# Autodesk Inventor assembly: spurgearTest
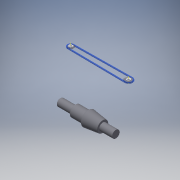
[picture p0: Inventor's stored thumbnail of the model, 180x180]
Saved by Autodesk Inventor 2016 (Build 200138000, 138)
## iProperties
Created: 2016-04-25
Part Number: spurgearTest
Document SubType Name: Assembly
Designer: Henrik Samuelsson
Author: Henrik Samuelsson
## Documents named in this file (4)
- C:\Users\Henrik Samuelsson\Documents\Killer-Bot-2016\AutodeskWorkspace\spurgearTest.iam
- C:\Users\Henrik Samuelsson\Documents\Killer-Bot-2016\AutodeskWorkspace\mountingHub6mm.ipt
- C:\Users\Henrik Samuelsson\Documents\Killer-Bot-2016\AutodeskWorkspace\spurgearTest\Design Accelerator\Shaft1.iam
- C:\Users\Henrik Samuelsson\Documents\Killer-Bot-2016\AutodeskWorkspace\spurgearTest\Design Accelerator\Chain Drive2.iam
## Components (4 placed, 3 different names)
1. mountingHub6mm:1 — Flush:1, Mate:2
2. mountingHub6mm:2 — Flush:1, Mate:1
3. Shaft:1 [sub-assembly]
4. Chain Drive:1 [sub-assembly] — Mate:1, Mate:2
## Relationships (3: Mate 2, Flush 1)
- Flush:1: mountingHub6mm:1 ↔ mountingHub6mm:2
- Mate:1: mountingHub6mm:2 ↔ Chain Drive:1
- Mate:2: mountingHub6mm:1 ↔ Chain Drive:1
